# Autodesk Inventor assembly: COXA_ROLL_LINK_ASM
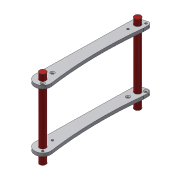
[picture p0: Inventor's stored thumbnail of the model, 180x180]
Saved by Autodesk Inventor 2019.4 (Build 234330000, 330)
## iProperties
Created: 2019-11-06
Part Number: COXA_ROLL_LINK_ASM
Material: 一般
Document SubType Name: Assembly
Designer: y6tada
Author: y6tada
## Documents named in this file (4)
- C:\Workspace\Yuni9\Inventor\Asm\COXA_UNIT\COXA_ROLL_LINK_ASM.iam
- C:\Workspace\Yuni9\Inventor\Asm\COXA_UNIT\COXA_ROLL_LONG-LINK.ipt
- C:\Workspace\Yuni9\Inventor\Asm\COXA_UNIT\COXA_ROLL_SHAFT_D4.ipt
- C:\Workspace\Yuni9\Inventor\Asm\COXA_UNIT\COXA_ROLL_LONG-LINK_MIR.ipt
## Components (4 placed, 3 different names)
1. COXA_ROLL_LONG-LINK:1 — フラッシュ:1, フラッシュ:2, メイト:1, メイト:2, フラッシュ:3
2. COXA_ROLL_SHAFT_D4:1 — メイト:1, フラッシュ:4, メイト:4
3. COXA_ROLL_SHAFT_D4:2 — メイト:2, フラッシュ:5, メイト:5
4. COXA_ROLL_LONG-LINK_MIR:1 — メイト:3, メイト:4, メイト:5
## Relationships (10: Flush 5, Mate 5)
- フラッシュ:1 [Flush]: COXA_ROLL_LONG-LINK:1
- フラッシュ:2 [Flush]: COXA_ROLL_LONG-LINK:1
- メイト:1 [Mate]: COXA_ROLL_LONG-LINK:1 ↔ COXA_ROLL_SHAFT_D4:1
- メイト:2 [Mate]: COXA_ROLL_LONG-LINK:1 ↔ COXA_ROLL_SHAFT_D4:2
- フラッシュ:3 [Flush] (19 mm): COXA_ROLL_LONG-LINK:1
- フラッシュ:4 [Flush]: COXA_ROLL_SHAFT_D4:1
- フラッシュ:5 [Flush]: COXA_ROLL_SHAFT_D4:2
- メイト:3 [Mate] (19 mm): COXA_ROLL_LONG-LINK_MIR:1
- メイト:4 [Mate]: COXA_ROLL_SHAFT_D4:1 ↔ COXA_ROLL_LONG-LINK_MIR:1
- メイト:5 [Mate]: COXA_ROLL_SHAFT_D4:2 ↔ COXA_ROLL_LONG-LINK_MIR:1
